# Autodesk Inventor assembly: Plasma-vacuum-vessel-152IC-cross-L205p8
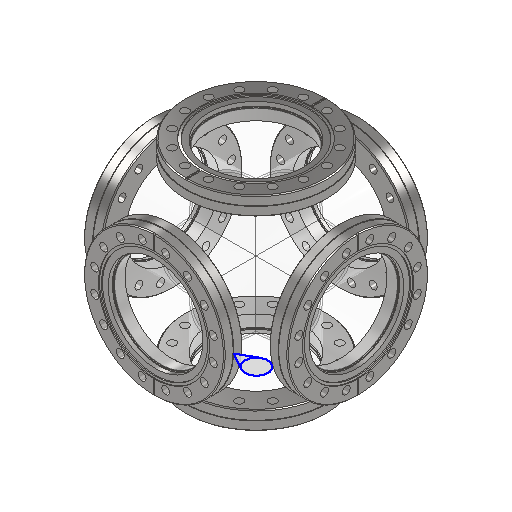
[picture p0: Inventor's stored thumbnail of the model, 512x512]
Saved by Autodesk Inventor 2026.2 (Build 302298000, 298)
## iProperties
Created: 2019-06-03
Part Number: Plasma-vacuum-vessel-152IC-cross-L205p8
Document SubType Name: Assembly
Designer: kuzmin
Mass: 9923.03 g
Surface Area: 5745.69 cm^2
Volume: 1272.81 cm^3
Density: 7.79613 g/cm^3
Author: kuzmin
## Documents named in this file (4)
- D:\repos\PIHTI\Plasma Vessel_1\PIHTI-for-boron_1\parts\Plasma-vacuum-vessel\Plasma-vacuum-vessel-152IC-cross-L205p8.iam
- D:\repos\PIHTI\Plasma Vessel\Plasma-vacuum-cross\UFC-152.ipt
- C:\Users\queez\Dropbox\Drawings\PIHTI\Plasma Vessel\Plasma-vacuum-cross\UFC.ipt
- D:\repos\PIHTI\Plasma Vessel_1\PIHTI-for-boron_1\parts\Plasma-vacuum-vessel\Cross-6way-152IC-L205p8.ipt
## Components (7 placed, 2 different names)
1. Cross-6way-152IC-L205p8:1 — フラッシュ:1, メイト:1, フラッシュ:2, リジッド:1, リジッド:3, リジッド:4, リジッド:2, リジッド:5, リジッド:6
2. UFC-152:1 — リジッド:3
3. UFC-152:2 — リジッド:4
4. UFC-152:3 — リジッド:2
5. UFC-152:4 — リジッド:6
6. UFC-152:5 — リジッド:1
7. UFC-152:6 — リジッド:5
## Relationships (9: WeldJoint 6, Flush 2, Mate 1)
- フラッシュ:1 [Flush]: Cross-6way-152IC-L205p8:1
- メイト:1 [Mate]: Cross-6way-152IC-L205p8:1
- フラッシュ:2 [Flush]: Cross-6way-152IC-L205p8:1
- リジッド:1 [WeldJoint]: Cross-6way-152IC-L205p8:1 ↔ UFC-152:5
- リジッド:3 [WeldJoint]: Cross-6way-152IC-L205p8:1 ↔ UFC-152:1
- リジッド:4 [WeldJoint]: Cross-6way-152IC-L205p8:1 ↔ UFC-152:2
- リジッド:2 [WeldJoint]: Cross-6way-152IC-L205p8:1 ↔ UFC-152:3
- リジッド:5 [WeldJoint]: Cross-6way-152IC-L205p8:1 ↔ UFC-152:6
- リジッド:6 [WeldJoint]: Cross-6way-152IC-L205p8:1 ↔ UFC-152:4
